# Autodesk Inventor assembly: Heater Connection Flange w/ rod
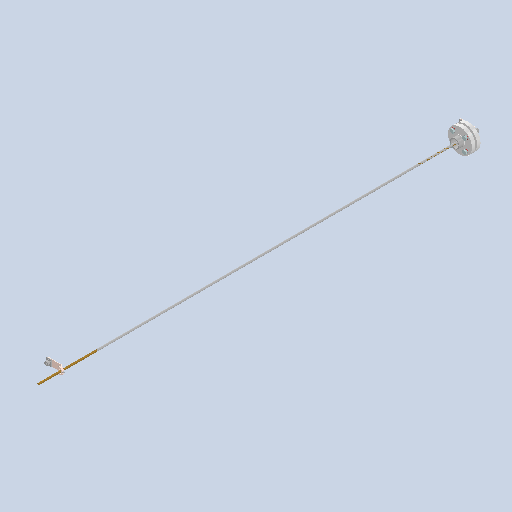
[picture p0: Inventor's stored thumbnail of the model, 512x512]
Saved by Autodesk Inventor 2027 (Build 310192000, 192)
## iProperties
Created: 2026-07-30
Part Number: Heater Connection Flange w/ rod
Document SubType Name: Assembly
Designer: AdminForWorker
Title: Heater Connection Flange w/ rod v8
Author: AdminForWorker
## Documents named in this file (20)
- C:\Users\ig2\Desktop\SMR Thermal\thermal-loop\resources\v0.1.2\CAD\Inventor\aa FINAL MODEL with proportional valve\Heater Connection Flange w_ rod v8.iam
- C:\Users\ig2\Desktop\SMR Thermal\thermal-loop\resources\v0.1.2\CAD\Inventor\aa FINAL MODEL with proportional valve\1 1_2 Silver Flange v2.ipt
- C:\Users\ig2\Desktop\SMR Thermal\thermal-loop\resources\v0.1.2\CAD\Inventor\aa FINAL MODEL with proportional valve\average flange blue seal v5.ipt
- C:\Users\ig2\Desktop\SMR Thermal\thermal-loop\resources\v0.1.2\CAD\Inventor\aa FINAL MODEL with proportional valve\average flange pipe v3.ipt
- C:\Users\ig2\Desktop\SMR Thermal\thermal-loop\resources\v0.1.2\CAD\Inventor\aa FINAL MODEL with proportional valve\bottom right silver connection flange v3.ipt
- C:\Users\ig2\Desktop\SMR Thermal\thermal-loop\resources\v0.1.2\CAD\Inventor\aa FINAL MODEL with proportional valve\bottom right heater connection v2.iam
- C:\Users\ig2\Desktop\SMR Thermal\thermal-loop\resources\v0.1.2\CAD\Inventor\aa FINAL MODEL with proportional valve\Thermal Nycrome Rod v1.ipt
- C:\Users\ig2\Desktop\SMR Thermal\thermal-loop\resources\v0.1.2\CAD\Inventor\aa FINAL MODEL with proportional valve\Coppor clamp to heater v2.ipt
- C:\Users\ig2\Desktop\SMR Thermal\thermal-loop\resources\v0.1.2\CAD\Inventor\aa FINAL MODEL with proportional valve\Top Hat Grommet v3.ipt
- C:\Users\ig2\Desktop\SMR Thermal\thermal-loop\resources\v0.1.2\CAD\Inventor\aa FINAL MODEL with proportional valve\1_2 in bolt v2.ipt
- C:\Users\ig2\Desktop\SMR Thermal\thermal-loop\resources\v0.1.2\CAD\Inventor\aa FINAL MODEL with proportional valve\1_2 in nut v2.ipt
- C:\Users\ig2\Desktop\SMR Thermal\thermal-loop\resources\v0.1.2\CAD\Inventor\aa FINAL MODEL with proportional valve\1_2 in washer narrow v2.iam
- C:\Users\ig2\Desktop\SMR Thermal\thermal-loop\resources\v0.1.2\CAD\Inventor\aa FINAL MODEL with proportional valve\1_2 in washer narrow v2_1.iam
- C:\Users\ig2\Desktop\SMR Thermal\thermal-loop\resources\v0.1.2\CAD\Inventor\aa FINAL MODEL with proportional valve\1_2 in washer narrow v2_2.iam
- C:\Users\ig2\Desktop\SMR Thermal\thermal-loop\resources\v0.1.2\CAD\Inventor\aa FINAL MODEL with proportional valve\1_2 in washer narrow v2_3.iam
- C:\Users\ig2\Desktop\SMR Thermal\thermal-loop\resources\v0.1.2\CAD\Inventor\aa FINAL MODEL with proportional valve\1_2 in washer narrow v2_4.iam
- C:\Users\ig2\Desktop\SMR Thermal\thermal-loop\resources\v0.1.2\CAD\Inventor\aa FINAL MODEL with proportional valve\1_2 in washer narrow v2_5.iam
- C:\Users\ig2\Desktop\SMR Thermal\thermal-loop\resources\v0.1.2\CAD\Inventor\aa FINAL MODEL with proportional valve\1_2 in washer narrow v2_6.iam
- C:\Users\ig2\Desktop\SMR Thermal\thermal-loop\resources\v0.1.2\CAD\Inventor\aa FINAL MODEL with proportional valve\1_2 in washer narrow v2_7.iam
- C:\Users\ig2\Downloads\2575T24_Tight-Tolerance Ultra-Machinable 360 Brass\2575T24_Tight-Tolerance Ultra-Machinable 360 Brass.ipt
## Components (33 placed, 12 different names)
1. 1 1/2 Silver Flange v2:1
2. average flange blue seal v5:1
3. average flange pipe v3:1
4. bottom right silver connection flange v3:1
5. bottom right heater connection v2:1 [sub-assembly]
6. Thermal Nycrome Rod v1:1 — Rotational:1, Rotational:2
7. Coppor clamp to heater v2:1
8. Top Hat Grommet v3:1
9. Top Hat Grommet v3:2
10. 1/2 in bolt v2:1
11. 1/2 in nut v2:1
12. 1/2 in washer narrow v2:1 [sub-assembly]
13. 1/2 in washer narrow v2:2 [sub-assembly]
14. Top Hat Grommet v3:3
15. Top Hat Grommet v3:4
16. 1/2 in washer narrow v2:3 [sub-assembly]
17. 1/2 in nut v2:2
18. 1/2 in bolt v2:2
19. 1/2 in washer narrow v2:4 [sub-assembly]
20. Top Hat Grommet v3:5
21. Top Hat Grommet v3:6
22. 1/2 in washer narrow v2:5 [sub-assembly]
23. 1/2 in nut v2:3
24. 1/2 in bolt v2:3
25. 1/2 in washer narrow v2:6 [sub-assembly]
26. Top Hat Grommet v3:7
27. Top Hat Grommet v3:8
28. 1/2 in washer narrow v2:7 [sub-assembly]
29. 1/2 in nut v2:4
30. 1/2 in bolt v2:4
31. 1/2 in washer narrow v2:8 [sub-assembly]
32. 2575T24_Tight-Tolerance Ultra-Machinable 360 Brass:1 — Rotational:2
33. 2575T24_Tight-Tolerance Ultra-Machinable 360 Brass:2 — Rotational:1
## Relationships (2: RevoluteJoint 2)
- Rotational:1 [RevoluteJoint]: Thermal Nycrome Rod v1:1 ↔ 2575T24_Tight-Tolerance Ultra-Machinable 360 Brass:2
- Rotational:2 [RevoluteJoint]: Thermal Nycrome Rod v1:1 ↔ 2575T24_Tight-Tolerance Ultra-Machinable 360 Brass:1
